# Autodesk Inventor assembly: sinkFrame
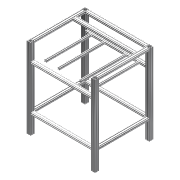
[picture p0: Inventor's stored thumbnail of the model, 180x180]
Saved by Autodesk Inventor 2018 (Build 220112000, 112)
## iProperties
Created: 2018-01-07
Part Number: sinkFrame
Document SubType Name: Assembly
Designer: sawaiz
Author: sawaiz
## Documents named in this file (4)
- C:\Users\sawaiz\OneDrive\personal\berlin\Move\larkspur\kitchen\frame\extrusions\sinkFrame.iam
- C:\Users\sawaiz\OneDrive\personal\berlin\Move\larkspur\kitchen\frame\extrusions\plate.iam
- C:\Users\sawaiz\OneDrive\personal\berlin\Move\larkspur\kitchen\frame\extrusions\HFS5-2040-600.ipt
- C:\Users\sawaiz\OneDrive\personal\berlin\Move\larkspur\kitchen\frame\extrusions\HFS5-2020-450.ipt
## Components (12 placed, 3 different names)
1. plate:1 [sub-assembly] — Flush:1, Flush:2, Mate:1, Flush:3, Flush:4, Symmetry:1, Symmetry:2, Symmetry:3
2. plate:2 [sub-assembly] — Flush:1, Flush:2, Mate:2, Mate:3, Flush:5, Mate:4, Flush:6, Flush:7, Flush:8, Mate:5, Flush:9, Flush:10, Flush:12, Mate:6, Flush:21, Mate:8, Flush:22, Symmetry:1, Symmetry:2, Symmetry:3
3. HFS5-2040-600:1 — Mate:1, Flush:3, Flush:4, Mate:2
4. HFS5-2040-600:2 — Flush:8, Mate:5, Flush:9
5. HFS5-2040-600:3 — Mate:4, Flush:6, Flush:7
6. HFS5-2040-600:4 — Mate:3, Flush:5, Flush:10, Flush:11
7. HFS5-2040-600:5 — Flush:11, Flush:12, Mate:6, Flush:13, Mate:7, Flush:20
8. HFS5-2020-450:1 — Flush:15, Flush:16, Flush:17, Flush:18, Flush:19
9. HFS5-2020-450:2 — Flush:16, Flush:17
10. HFS5-2020-450:3 — Flush:14, Flush:19, Mate:7, Flush:20
11. HFS5-2020-450:4 — Flush:13, Flush:14, Flush:15, Flush:18
12. HFS5-2040-600:6 — Flush:21, Mate:8, Flush:22
## Relationships (33: Flush 22, Mate 8, Symmetry 3)
- Flush:1: plate:1 ↔ plate:2
- Flush:2: plate:1 ↔ plate:2
- Mate:1: plate:1 ↔ HFS5-2040-600:1
- Flush:3: plate:1 ↔ HFS5-2040-600:1
- Flush:4: plate:1 ↔ HFS5-2040-600:1
- Mate:2: plate:2 ↔ HFS5-2040-600:1
- Mate:3: plate:2 ↔ HFS5-2040-600:4
- Flush:5: plate:2 ↔ HFS5-2040-600:4
- Mate:4: plate:2 ↔ HFS5-2040-600:3
- Flush:6: plate:2 ↔ HFS5-2040-600:3
- Flush:7: plate:2 ↔ HFS5-2040-600:3
- Flush:8: plate:2 ↔ HFS5-2040-600:2
- Mate:5: plate:2 ↔ HFS5-2040-600:2
- Flush:9: plate:2 ↔ HFS5-2040-600:2
- Flush:10 (162 mm): plate:2 ↔ HFS5-2040-600:4
- Flush:11: HFS5-2040-600:4 ↔ HFS5-2040-600:5
- Flush:12: plate:2 ↔ HFS5-2040-600:5
- Mate:6: plate:2 ↔ HFS5-2040-600:5
- Flush:13: HFS5-2040-600:5 ↔ HFS5-2020-450:4
- Flush:14: HFS5-2020-450:3 ↔ HFS5-2020-450:4
- Flush:15: HFS5-2020-450:1 ↔ HFS5-2020-450:4
- Flush:16: HFS5-2020-450:1 ↔ HFS5-2020-450:2
- Flush:17: HFS5-2020-450:1 ↔ HFS5-2020-450:2
- Flush:18: HFS5-2020-450:1 ↔ HFS5-2020-450:4
- Flush:19: HFS5-2020-450:1 ↔ HFS5-2020-450:3
- Mate:7: HFS5-2040-600:5 ↔ HFS5-2020-450:3
- Flush:20: HFS5-2040-600:5 ↔ HFS5-2020-450:3
- Flush:21: plate:2 ↔ HFS5-2040-600:6
- Mate:8: plate:2 ↔ HFS5-2040-600:6
- Flush:22 (420 mm): plate:2 ↔ HFS5-2040-600:6
- Symmetry:1: plate:1 ↔ plate:2
- Symmetry:2: plate:1 ↔ plate:2
- Symmetry:3: plate:1 ↔ plate:2
